# Autodesk Inventor assembly: Tank_Tread_without_Rubber
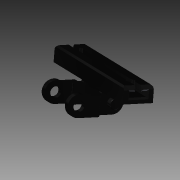
[picture p0: Inventor's stored thumbnail of the model, 180x180]
Saved by Autodesk Inventor 2015 (Build 190159000, 159)
## iProperties
Created: 2015-10-14
Part Number: Tank_Tread_without_Rubber
Document SubType Name: Assembly
Designer: nojessen
Author: nojessen
## Documents named in this file (4)
- C:\Users\nojessen\Documents\GitHub\CAD\COTSParts\Tetrix\Tank Treads\Tank_Tread_without_Rubber.iam
- C:\Users\nojessen\Documents\GitHub\CAD\COTSParts\Tetrix\Tank Treads\TETRIX_TT_LINK_1_2011.ipt
- C:\Users\nojessen\Documents\GitHub\CAD\COTSParts\Tetrix\Tank Treads\TETRIX_TT_LINK_2_2011.ipt
- C:\Users\nojessen\Documents\GitHub\CAD\COTSParts\Tetrix\Tank Treads\TETRIX_TT_LINK_4_2011.ipt
## Components (3 placed, 3 different names)
1. TETRIX_TT_LINK_1_2011:1 — Mate:1, Mate:2, Flush:1, Mate:5
2. TETRIX_TT_LINK_2_2011:1 — Mate:3, Mate:4, Flush:1
3. TETRIX_TT_LINK_4_2011:1 — Mate:1, Mate:2, Mate:3, Mate:4, Mate:5
## Relationships (6: Mate 5, Flush 1)
- Mate:1: TETRIX_TT_LINK_1_2011:1 ↔ TETRIX_TT_LINK_4_2011:1
- Mate:2: TETRIX_TT_LINK_1_2011:1 ↔ TETRIX_TT_LINK_4_2011:1
- Mate:3: TETRIX_TT_LINK_2_2011:1 ↔ TETRIX_TT_LINK_4_2011:1
- Mate:4: TETRIX_TT_LINK_2_2011:1 ↔ TETRIX_TT_LINK_4_2011:1
- Flush:1: TETRIX_TT_LINK_1_2011:1 ↔ TETRIX_TT_LINK_2_2011:1
- Mate:5: TETRIX_TT_LINK_1_2011:1 ↔ TETRIX_TT_LINK_4_2011:1
